# Autodesk Inventor assembly: Gripper Attempt 01
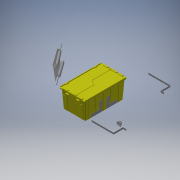
[picture p0: Inventor's stored thumbnail of the model, 180x180]
Saved by Autodesk Inventor 2016 (Build 200138000, 138)
## iProperties
Created: 2015-06-18
Part Number: Gripper Attempt 01
Document SubType Name: Assembly
Designer: steele
Author: steele
## Documents named in this file (11)
- C:\snobotics\CAD\robSteele\Gripper\Gripper Attempt 01.iam
- C:\snobotics\CAD\partResources\AutodeskParts\2015\FRC_FieldModel_2015\Parts\YELLOW_TOTEASM_ASM.iam
- C:\snobotics\CAD\robSteele\ipart Components\Plot for Gripper.ipt
- C:\snobotics\CAD\robSteele\ipart Components\Rail For Gripper.ipt
- C:\snobotics\CAD\robSteele\ipart Components\Rail For Gripper\Rail For Gripper 1 x 12 x 3_16.ipt
- C:\snobotics\CAD\robSteele\ipart Components\Gripper Arm\Gripper Arm-01.ipt
- C:\snobotics\CAD\robSteele\ipart Components\Gripper Arm.ipt
- C:\snobotics\CAD\partResources\McMaster-Carr\Air Cylinder\Pivot Mount Cylinders\Pivot Bracket for 1_50 Bore\6498K730.ipt
- C:\snobotics\CAD\partResources\McMaster-Carr\Air Cylinder\Pivot Mount Cylinders\Single Acting With Spring Return\Force 155 Bore 1_50\Stroke 12\6498K786.ipt
- C:\snobotics\CAD\robSteele\ipart Components\Plot for Gripper\Plate for Gripper 8 x 27 x 1_4.ipt
- C:\snobotics\CAD\partResources\McMaster-Carr\Air Cylinder\Pivot Mount Cylinders\Foot Bracket for 1_25 and 1_50 Bore\6498K340.ipt
## Components (12 placed, 7 different names)
1. YELLOW_TOTEASM_ASM:1 [sub-assembly]
2. Plate for Gripper 8 x 27 x 1_4:1 — Flush:1, Mate:1, Flush:2, Mate:2, Flush:3, Flush:4, Mate:3, Flush:5, Flush:6, Mate:4, Flush:7, Flush:8, Mate:5
3. Rail For Gripper 1 x 12 x 3_16:1 — Flush:1, Mate:1, Flush:2
4. Rail For Gripper 1 x 12 x 3_16:2 — Mate:2, Flush:3, Flush:4
5. Gripper Arm-01:1
6. Gripper Arm-01:2
7. 6498K730:1 — Mate:3, Flush:5, Flush:6, Insert:2
8. 6498K730:2 — Mate:4, Flush:7, Flush:8, Insert:1, Flush:9
9. 6498K786:1 — Insert:2
10. 6498K786:2 — Insert:1
11. 6498K340:1
12. 6498K340:2 — Mate:5, Flush:9
## Relationships (16: Flush 9, Mate 5, Insert 2)
- Flush:1: Plate for Gripper 8 x 27 x 1_4:1 ↔ Rail For Gripper 1 x 12 x 3_16:1
- Mate:1: Plate for Gripper 8 x 27 x 1_4:1 ↔ Rail For Gripper 1 x 12 x 3_16:1
- Flush:2: Plate for Gripper 8 x 27 x 1_4:1 ↔ Rail For Gripper 1 x 12 x 3_16:1
- Mate:2: Plate for Gripper 8 x 27 x 1_4:1 ↔ Rail For Gripper 1 x 12 x 3_16:2
- Flush:3: Plate for Gripper 8 x 27 x 1_4:1 ↔ Rail For Gripper 1 x 12 x 3_16:2
- Flush:4: Plate for Gripper 8 x 27 x 1_4:1 ↔ Rail For Gripper 1 x 12 x 3_16:2
- Mate:3: Plate for Gripper 8 x 27 x 1_4:1 ↔ 6498K730:1
- Flush:5: Plate for Gripper 8 x 27 x 1_4:1 ↔ 6498K730:1
- Flush:6: Plate for Gripper 8 x 27 x 1_4:1 ↔ 6498K730:1
- Mate:4: Plate for Gripper 8 x 27 x 1_4:1 ↔ 6498K730:2
- Flush:7: Plate for Gripper 8 x 27 x 1_4:1 ↔ 6498K730:2
- Flush:8: Plate for Gripper 8 x 27 x 1_4:1 ↔ 6498K730:2
- Insert:1: 6498K730:2 ↔ 6498K786:2
- Insert:2: 6498K730:1 ↔ 6498K786:1
- Mate:5: Plate for Gripper 8 x 27 x 1_4:1 ↔ 6498K340:2
- Flush:9: 6498K730:2 ↔ 6498K340:2
